# Autodesk Inventor assembly: ASY PNS 1600 Filter column D1000
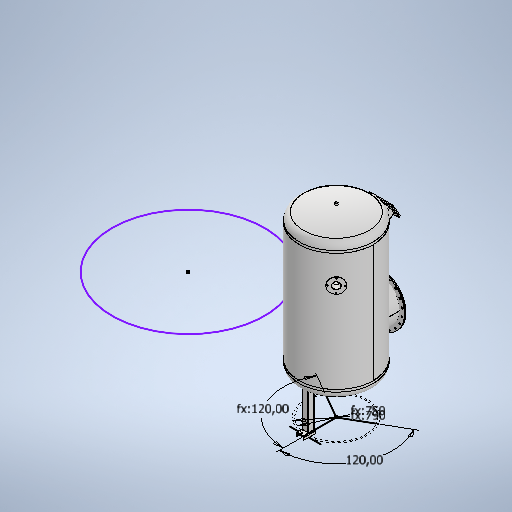
[picture p0: Inventor's stored thumbnail of the model, 512x512]
Saved by Autodesk Inventor 2025.3 (Build 293356030, 356C)
## iProperties
Created: 2025-02-13
Part Number: ASY PNS 1600 Filter column D1000
Document SubType Name: Assembly
Designer: pokla
Mass: 294380 g
Surface Area: 201489 cm^2
Volume: 65316.1 cm^3
Density: 4.50701 g/cm^3
allow_slope_adjustment: 0 ul
flow_configuration2: 1 ul
flow_direction: 2 ul
loss_method: 0 ul
radius: 45,500 mm
radius: 16,750 mm
Author: pokla
Revision Number: 3
## iProperties of the stored document MemberDocs/xS3xdvqv2Fs4urkfuOqhnp5u1Be
allow_slope_adjustment: 0 ul
flow_configuration2: 1 ul
flow_direction: 2 ul
loss_method: 0 ul
radius: 45,500 mm
Created: 2025-02-13
Part Number: ASY PNS 1600 Filter column D1000
Document SubType Name: Assembly
Designer: pokla
Mass: 294380 g
Surface Area: 201489 cm^2
Volume: 65316.1 cm^3
Density: 4.50701 g/cm^3
radius: 16,750 mm
Author: pokla
Revision Number: 3
## iProperties of the stored document MemberDocs/xVvj5wjhiIso5nm03Gzgds4hn2d
Created: 2025-02-13
Part Number: ASY PNS 1600 Filter column D1000
Document SubType Name: Assembly
Designer: pokla
Mass: 294380 g
Surface Area: 201489 cm^2
Volume: 65316.1 cm^3
Density: 4.50701 g/cm^3
allow_slope_adjustment: 0 ul
flow_configuration2: 1 ul
flow_direction: 2 ul
loss_method: 0 ul
radius: 45,500 mm
radius: 16,750 mm
Author: pokla
Revision Number: 3
## Documents named in this file (25)
- C:\Users\admin\Documents\Inventor\SLM-Salemal\ASY SLM 1600 Filter column D940.iam
- C:\Users\admin\Documents\Inventor\SLM-Salemal\PNS-612 accses hatch flangeipt.ipt
- C:\Users\admin\Documents\Inventor\SLM-Salemal\PNS-611 accses hatch tube.ipt
- C:\Users\admin\Documents\Inventor\SLM-Salemal\PNS 1602 main Shell D1000.ipt
- C:\Users\admin\Documents\Inventor\SLM-Salemal\PNS 1604 dished head D1000.ipt
- C:\Users\admin\Documents\Inventor\SLM-Salemal\Fitting G1.ipt
- C:\Users\admin\Documents\Inventor\SLM-Salemal\ASY PNS 1690 Filter legs D1000.iam
- C:\Users\admin\Documents\Inventor\SLM-Salemal\PNS 1633 charging blind flange.ipt
- C:\Users\admin\Documents\Inventor\SLM-Salemal\ASY PNS 1610 charging hatch.iam
- C:\Users\admin\Documents\Inventor\SLM-Salemal\cc\JIS B 2312 90 Deg Long Elbow Steel 80A x Sch 40.ipt
- C:\Users\admin\Documents\Inventor\SLM-Salemal\ASY PNS 1650 filter-distribution-system 1000.iam
- C:\Users\admin\Documents\Inventor\SLM-Salemal\PNS 1612 FDS tube 2.ipt
- C:\Users\admin\Documents\Inventor\SLM-Salemal\PNS 1606 charging flange round.ipt
- C:\Users\admin\Documents\Inventor\SLM-Salemal\PNS 1613 FDS tube 3.ipt
- C:\Users\admin\Documents\Inventor\SLM-Salemal\PNS 1614 FDS tube 4.ipt
- C:\Users\admin\Documents\Inventor\SLM-Salemal\PNS 1615 FDS tube 5.ipt
- C:\Users\admin\Documents\Inventor\SLM-Salemal\ASY PNS 179 top funnel 1200 50-90_1000x90.iam
- C:\Users\admin\Documents\Inventor\SLM-Salemal\pallet jack dummy.ipt
- C:\Users\admin\Documents\Inventor\SLM-Salemal\SLM 1431 FDS flange DN90.ipt
- C:\Users\admin\Documents\Inventor\SLM-Salemal\SLM 1432 FDS free flange DN90.ipt
- C:\Users\admin\Documents\Inventor\SLM-Salemal\SLM 1671 charging tube 1.ipt
- C:\Users\admin\Documents\Inventor\SLM-Salemal\SLM 1672 charging tube 2.ipt
- C:\Users\admin\Documents\Inventor\SLM-Salemal\PNS 1607 charging flange rect.ipt
- C:\Users\admin\Documents\Inventor\SLM-Salemal\PNS 9110 main Shell D 940.ipt
- C:\Users\admin\Documents\Inventor\SLM-Salemal\SLM 1601 DIM Filter column D940.ipt
## Components (28 placed, 24 different names)
1. PNS 1602 main Shell D1000.ipt:1 — Rigid:10, Rigid:13, Rigid:14, Mate:1, Mate:2, Rigid:74, Rigid:80
2. Fitting G1.ipt:1 — Rigid:15
3. PNS 1633 charging blind flange.ipt:2 — Rigid:67
4. ASY PNS 1650 filter-distribution-system 1000.iam:1 [sub-assembly] — Rotational:75
5. ASY PNS 179 top funnel 1200 50-90_1000x90:1 [sub-assembly] — Rotational:72
6. pallet jack dummy:1
7. PNS 1633 charging blind flange:5 — Rigid:77
8. PNS 1633 charging blind flange:6 — Rigid:78, Rotational:72
9. PNS 1604 dished head D1000.ipt:1 — Rigid:13, Rigid:75
10. Fitting G1.ipt:2
11. JIS B 2312 90 Deg Long Elbow Steel 80A x Sch 40.ipt:1 — Rigid:68, Rigid:79
12. PNS 1613 FDS tube 3:1 — Rigid:67, Rigid:68
13. PNS 1614 FDS tube 4:1 — Rigid:79, Rigid:75, Rotational:71, Rotational:75
14. SLM 1431 FDS flange DN90:1 — Rigid:76
15. SLM 1432 FDS free flange DN90:1 — Rotational:71, Rigid:76
16. PNS-611 accses hatch tube.ipt:1 — Rigid:10, Rotational:74
17. PNS 1604 dished head D1000.ipt:2 — Rigid:14, Rigid:15, Mate:3
18. JIS B 2312 90 Deg Long Elbow Steel 80A x Sch 40.ipt:2 — Rigid:62, Rigid:73
19. PNS 1612 FDS tube 2:3 — Rigid:62, Rigid:78
20. PNS 1615 FDS tube 5:1 — Rigid:73, Rigid:74, Rigid:77
21. SLM 1672 charging tube 2:1 — Rigid:82, Rigid:84
22. SLM 1671 charging tube 1:1 — Rigid:80, Rigid:84
23. PNS 1606 charging flange round:1 — Rigid:82, Rigid:83
24. PNS 1607 charging flange rect:1 — Rigid:83
25. PNS-612 accses hatch flangeipt.ipt:1 — Rotational:73, Rotational:74
26. ASY PNS 1610 charging hatch.iam:1 [sub-assembly] — Rotational:73
27. ASY PNS 1690 Filter legs D1000.iam:1 [sub-assembly] — Flush:2, Mate:4, Mate:5
28. PNS 9110 main Shell D 940:1 — Mate:6, Mate:7
## Relationships (31: WeldJoint 18, Mate 7, RevoluteJoint 5, Flush 1)
- Rigid:10 [WeldJoint] (66 mm): PNS 1602 main Shell D1000.ipt:1 ↔ PNS-611 accses hatch tube.ipt:1
- Rigid:13 [WeldJoint]: PNS 1602 main Shell D1000.ipt:1 ↔ PNS 1604 dished head D1000.ipt:1
- Rigid:14 [WeldJoint]: PNS 1602 main Shell D1000.ipt:1 ↔ PNS 1604 dished head D1000.ipt:2
- Rigid:15 [WeldJoint]: Fitting G1.ipt:1 ↔ PNS 1604 dished head D1000.ipt:2
- Mate:1: PNS 1602 main Shell D1000.ipt:1
- Mate:2: PNS 1602 main Shell D1000.ipt:1
- Mate:3 (2350 mm): PNS 1604 dished head D1000.ipt:2
- Flush:2: ASY PNS 1690 Filter legs D1000.iam:1
- Rigid:62 [WeldJoint]: JIS B 2312 90 Deg Long Elbow Steel 80A x Sch 40.ipt:2 ↔ PNS 1612 FDS tube 2:3
- Rigid:67 [WeldJoint]: PNS 1633 charging blind flange.ipt:2 ↔ PNS 1613 FDS tube 3:1
- Rigid:68 [WeldJoint]: JIS B 2312 90 Deg Long Elbow Steel 80A x Sch 40.ipt:1 ↔ PNS 1613 FDS tube 3:1
- Rigid:79 [WeldJoint]: JIS B 2312 90 Deg Long Elbow Steel 80A x Sch 40.ipt:1 ↔ PNS 1614 FDS tube 4:1
- Rigid:73 [WeldJoint]: JIS B 2312 90 Deg Long Elbow Steel 80A x Sch 40.ipt:2 ↔ PNS 1615 FDS tube 5:1
- Rigid:74 [WeldJoint] (80 mm): PNS 1602 main Shell D1000.ipt:1 ↔ PNS 1615 FDS tube 5:1
- Rigid:75 [WeldJoint] (-50 mm): PNS 1604 dished head D1000.ipt:1 ↔ PNS 1614 FDS tube 4:1
- Rotational:71 [RevoluteJoint]: PNS 1614 FDS tube 4:1 ↔ SLM 1432 FDS free flange DN90:1
- Rigid:76 [WeldJoint]: SLM 1431 FDS flange DN90:1 ↔ SLM 1432 FDS free flange DN90:1
- Rigid:77 [WeldJoint]: PNS 1633 charging blind flange:5 ↔ PNS 1615 FDS tube 5:1
- Rigid:78 [WeldJoint]: PNS 1633 charging blind flange:6 ↔ PNS 1612 FDS tube 2:3
- Rotational:72 [RevoluteJoint]: ASY PNS 179 top funnel 1200 50-90_1000x90:1 ↔ PNS 1633 charging blind flange:6
- Rotational:73 [RevoluteJoint]: PNS-612 accses hatch flangeipt.ipt:1 ↔ ASY PNS 1610 charging hatch.iam:1
- Rotational:74 [RevoluteJoint]: PNS-611 accses hatch tube.ipt:1 ↔ PNS-612 accses hatch flangeipt.ipt:1
- Rotational:75 [RevoluteJoint]: ASY PNS 1650 filter-distribution-system 1000.iam:1 ↔ PNS 1614 FDS tube 4:1
- Rigid:80 [WeldJoint]: PNS 1602 main Shell D1000.ipt:1 ↔ SLM 1671 charging tube 1:1
- Rigid:82 [WeldJoint]: SLM 1672 charging tube 2:1 ↔ PNS 1606 charging flange round:1
- Rigid:83 [WeldJoint]: PNS 1606 charging flange round:1 ↔ PNS 1607 charging flange rect:1
- Rigid:84 [WeldJoint]: SLM 1672 charging tube 2:1 ↔ SLM 1671 charging tube 1:1
- Mate:4: ASY PNS 1690 Filter legs D1000.iam:1
- Mate:5: ASY PNS 1690 Filter legs D1000.iam:1
- Mate:6: PNS 9110 main Shell D 940:1
- Mate:7: PNS 9110 main Shell D 940:1
